# Autodesk Inventor assembly: Assembly2
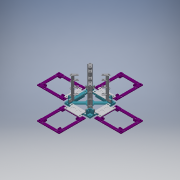
[picture p0: Inventor's stored thumbnail of the model, 180x180]
Saved by Autodesk Inventor 2016 (Build 200138000, 138)
## iProperties
Created: 2015-05-06
Part Number: Assembly2
Document SubType Name: Assembly
Designer: Erin
Mass: 23.6327 g
Surface Area: 477.241 cm^2
Volume: 37.8693 cm^3
Density: 0.62406 g/cm^3
Author: Erin
## Documents named in this file (21)
- C:\Users\Erin\Desktop\RDAS v0.2\Assembly.iam
- C:\Users\Erin\Desktop\RDAS v0.2\Base.ipt
- C:\Users\Erin\Desktop\RDAS v0.2\SideLink.ipt
- C:\Users\Erin\Desktop\RDAS v0.2\Side.ipt
- C:\Users\Erin\Desktop\RDAS v0.2\SideSizeAttach.ipt
- C:\Users\Erin\Desktop\RDAS v0.2\BaseVertical.ipt
- C:\Users\Erin\Desktop\RDAS v0.2\BaseSliders.ipt
- C:\Users\Erin\Desktop\RDAS v0.2\VerticalConnector_Longest.ipt
- C:\Users\Erin\Desktop\RDAS v0.2\SideTopper.ipt
- C:\Users\Erin\Desktop\RDAS v0.2\Assembly2\AIP\FEA\beta0vpy8.fins
- C:\Users\Erin\Desktop\RDAS v0.2\Assembly2\AIP\FEA\beta0vpz4.fsat
- C:\Users\Erin\Desktop\RDAS v0.2\Assembly2\AIP\FEA\beta0vpz4.ftes
- C:\Users\Erin\Desktop\RDAS v0.2\Assembly2\AIP\FEA\beta0vq00.fwiz
- C:\Users\Erin\Desktop\RDAS v0.2\Assembly2\AIP\FEA\beta0vq74.fmsh
- C:\Users\Erin\Desktop\RDAS v0.2\Assembly2\AIP\FEA\beta0vq80.fres
- C:\Users\Erin\Desktop\RDAS v0.2\Assembly2\AIP\FEA\bex3ksry8.fins
- C:\Users\Erin\Desktop\RDAS v0.2\Assembly2\AIP\FEA\bex3ksrz4.fsat
- C:\Users\Erin\Desktop\RDAS v0.2\Assembly2\AIP\FEA\bex3ksrz4.ftes
- C:\Users\Erin\Desktop\RDAS v0.2\Assembly2\AIP\FEA\bex3ksrz4.fwiz
- C:\Users\Erin\Desktop\RDAS v0.2\Assembly2\AIP\FEA\bex3ksskg.fmsh
- C:\Users\Erin\Desktop\RDAS v0.2\Assembly2\AIP\FEA\bex3ksslc.fres
## Components (17 placed, 8 different names)
1. Base:1 — Insert:1, Insert:2, Insert:3, Insert:4, Insert:5, Insert:6, Insert:7, Insert:8
2. SideLink:1 — Insert:1, Insert:4
3. SideLink:2 — Insert:5, Insert:6, Insert:9, Insert:10
4. SideLink:3 — Insert:7, Insert:8, Insert:15, Insert:16
5. SideLink:4 — Insert:2, Insert:3, Insert:13, Insert:14
6. Side:1
7. Side:2 — Insert:13, Insert:14
8. Side:3 — Insert:15, Insert:16
9. Side:4 — Insert:9, Insert:10
10. SideSizeAttach:1
11. BaseVertical:1
12. BaseSliders:1
13. VerticalConnector_Longest:1
14. VerticalConnector_Longest:2
15. VerticalConnector_Longest:3
16. VerticalConnector_Longest:4
17. SideTopper:1
## Relationships (14: Insert 14)
- Insert:1: Base:1 ↔ SideLink:1
- Insert:2: Base:1 ↔ SideLink:4
- Insert:3: Base:1 ↔ SideLink:4
- Insert:4: Base:1 ↔ SideLink:1
- Insert:5: Base:1 ↔ SideLink:2
- Insert:6: Base:1 ↔ SideLink:2
- Insert:7: Base:1 ↔ SideLink:3
- Insert:8: Base:1 ↔ SideLink:3
- Insert:9: SideLink:2 ↔ Side:4
- Insert:10: SideLink:2 ↔ Side:4
- Insert:13: SideLink:4 ↔ Side:2
- Insert:14: SideLink:4 ↔ Side:2
- Insert:15: SideLink:3 ↔ Side:3
- Insert:16: SideLink:3 ↔ Side:3
## Named parameters: sa_0 = 0, sa_1 = 0, sa_2 = 500, sa_3 = 5 mm, sa_4 = 5 mm, sa_6 = 5 mm, sa_5 = 5 mm, sa_7 = -3 mm, sa_8 = -3 mm, sa_9 = 0, sa_10 = 0, sa_11 = -100
note: some values were not read from the file. Shown as the stored number, unit unknown: "sa_0", "sa_1", "sa_2", "sa_9", "sa_10", "sa_11".
